# Autodesk Inventor assembly: InnerTopAssem
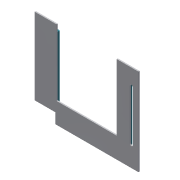
[picture p0: Inventor's stored thumbnail of the model, 180x180]
Saved by Autodesk Inventor 2014 (Build 180170000, 170)
## iProperties
Created: 2015-01-19
Part Number: InnerTopAssem
Document SubType Name: Assembly
Designer: Peele
Author: Peele
## Documents named in this file (4)
- E:\Copy\DLP\PandaPrint\SubAssem\InnerTopAssem.iam
- E:\Copy\DLP\PandaPrint\CustomParts\InnerTop.ipt
- E:\Copy\DLP\PandaPrint\StockParts\Rail.ipt
- E:\Copy\DLP\PandaPrint\StockParts\Rail\Rail-06.ipt
## Components (3 placed, 2 different names)
1. InnerTop:1 — Mate:1, Mate:2, Flush:1, Mate:3, Flush:6
2. Rail-06:1 — Mate:3, Flush:2, Flush:3, Flush:5
3. Rail-06:2 — Flush:2, Flush:4, Flush:5, Flush:6
## Relationships (9: Flush 6, Mate 3)
- Mate:1: InnerTop:1
- Mate:2: InnerTop:1
- Flush:1: InnerTop:1
- Mate:3: InnerTop:1 ↔ Rail-06:1
- Flush:2: Rail-06:1 ↔ Rail-06:2
- Flush:3 (87.5 mm): Rail-06:1
- Flush:4 (-87.5 mm): Rail-06:2
- Flush:5: Rail-06:1 ↔ Rail-06:2
- Flush:6 (25 mm): InnerTop:1 ↔ Rail-06:2
